# Autodesk Inventor assembly: 20-J2
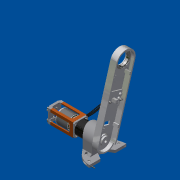
[picture p0: Inventor's stored thumbnail of the model, 180x180]
Saved by Autodesk Inventor 2018 (Build 220112000, 112)
## iProperties
Created: 2020-01-14
Part Number: 20-J2
Document SubType Name: Assembly
Designer: Bunny320
Author: Bunny320
## Documents named in this file (10)
- C:\Users\Bunny320\Desktop\sechs\4-CAD\20-J2.iam
- C:\Users\Bunny320\Desktop\sechs\4-CAD\201-flange-with motor.ipt
- C:\Users\Bunny320\Desktop\sechs\4-CAD\standardParts\61807-2RS1\61807-2RS1.iam
- C:\Users\Bunny320\Desktop\sechs\4-CAD\motor unit.iam
- C:\Users\Bunny320\Desktop\sechs\4-CAD\203-link left.ipt
- C:\Users\Bunny320\Desktop\sechs\4-CAD\standardParts\W 638_3-2Z\W 638_3-2Z.iam
- C:\Users\Bunny320\Documents\Inventor\Content Center Files\R2018\en-US\ISO 10642(2)\ISO 10642  - M4  x  20.ipt
- C:\Users\Bunny320\Documents\Inventor\Content Center Files\R2018\en-US\ISO 4762(1)\DIN EN ISO 4762 - M3 x 12.ipt
- C:\Users\Bunny320\Documents\Inventor\Content Center Files\R2018\en-US\ISO 4762(1)\DIN EN ISO 4762 - M3 x 20.ipt
- C:\Users\Bunny320\Documents\Inventor\Content Center Files\R2018\en-US\DIN EN ISO 4032\DIN EN ISO 4032 - M3.ipt
## Components (19 placed, 9 different names)
1. 201-flange-with motor:1 — Flush:1, Flush:2, Flush:3, Mate:3, Mate:4, Mate:7, Mate:8, Mate:9, Mate:21, Mate:22, Mate:23, Mate:24, Mate:31, Mate:32, Mate:33, Mate:34, Mate:35, Mate:36, Mate:37, Mate:38, Mate:39, Mate:40, Mate:41, Mate:42
2. 61807-2RS1:1 [sub-assembly] — Mate:3, Mate:4, Mate:14
3. motor unit:1 [sub-assembly] — Mate:7, Mate:8, Mate:9, Mate:13
4. 203-link left:1 — Mate:13, Mate:14, Mate:15, Mate:16, Mate:17, Mate:18, Mate:19, Mate:20, Mate:25, Mate:29
5. 61807-2RS1:3 [sub-assembly] — Mate:15, Mate:16
6. W 638_3-2Z:1 [sub-assembly] — Mate:17, Mate:20, Mate:26, Mate:30
7. W 638_3-2Z:2 [sub-assembly] — Mate:18, Mate:19
8. DIN EN ISO 10642 M4  x  20:1 — Mate:21
9. DIN EN ISO 10642 M4  x  20:2 — Mate:22
10. DIN EN ISO 10642 M4  x  20:3 — Mate:23
11. DIN EN ISO 10642 M4  x  20:4 — Mate:24
12. DIN EN ISO 4762 M3 x 12:1 — Mate:25, Mate:26
13. DIN EN ISO 4762 M3 x 12:3 — Mate:29, Mate:30
14. DIN EN ISO 4762 M3 x 12:4 — Mate:31, Mate:32
15. DIN EN ISO 4762 M3 x 12:5 — Mate:33, Mate:34
16. DIN EN ISO 4762 M3 x 12:6 — Mate:35, Mate:36
17. DIN EN ISO 4762 M3 x 12:7 — Mate:37, Mate:38
18. DIN EN ISO 4762 M3 x 20:1 — Mate:39, Mate:40
19. DIN EN ISO 4032 M3:1 — Mate:41, Mate:42
## Relationships (36: Mate 33, Flush 3)
- Flush:1: 201-flange-with motor:1
- Flush:2: 201-flange-with motor:1
- Flush:3: 201-flange-with motor:1
- Mate:3: 201-flange-with motor:1 ↔ 61807-2RS1:1
- Mate:4: 201-flange-with motor:1 ↔ 61807-2RS1:1
- Mate:7: 201-flange-with motor:1 ↔ motor unit:1
- Mate:8: 201-flange-with motor:1 ↔ motor unit:1
- Mate:9: 201-flange-with motor:1 ↔ motor unit:1
- Mate:13: motor unit:1 ↔ 203-link left:1
- Mate:14: 61807-2RS1:1 ↔ 203-link left:1
- Mate:15: 203-link left:1 ↔ 61807-2RS1:3
- Mate:16: 203-link left:1 ↔ 61807-2RS1:3
- Mate:17: 203-link left:1 ↔ W 638_3-2Z:1
- Mate:18: 203-link left:1 ↔ W 638_3-2Z:2
- Mate:19: 203-link left:1 ↔ W 638_3-2Z:2
- Mate:20: 203-link left:1 ↔ W 638_3-2Z:1
- Mate:21: 201-flange-with motor:1 ↔ DIN EN ISO 10642 M4  x  20:1
- Mate:22: 201-flange-with motor:1 ↔ DIN EN ISO 10642 M4  x  20:2
- Mate:23: 201-flange-with motor:1 ↔ DIN EN ISO 10642 M4  x  20:3
- Mate:24: 201-flange-with motor:1 ↔ DIN EN ISO 10642 M4  x  20:4
- Mate:25: 203-link left:1 ↔ DIN EN ISO 4762 M3 x 12:1
- Mate:26: W 638_3-2Z:1 ↔ DIN EN ISO 4762 M3 x 12:1
- Mate:29: 203-link left:1 ↔ DIN EN ISO 4762 M3 x 12:3
- Mate:30: W 638_3-2Z:1 ↔ DIN EN ISO 4762 M3 x 12:3
- Mate:31: 201-flange-with motor:1 ↔ DIN EN ISO 4762 M3 x 12:4
- Mate:32: 201-flange-with motor:1 ↔ DIN EN ISO 4762 M3 x 12:4
- Mate:33: 201-flange-with motor:1 ↔ DIN EN ISO 4762 M3 x 12:5
- Mate:34: 201-flange-with motor:1 ↔ DIN EN ISO 4762 M3 x 12:5
- Mate:35: 201-flange-with motor:1 ↔ DIN EN ISO 4762 M3 x 12:6
- Mate:36: 201-flange-with motor:1 ↔ DIN EN ISO 4762 M3 x 12:6
- Mate:37: 201-flange-with motor:1 ↔ DIN EN ISO 4762 M3 x 12:7
- Mate:38: 201-flange-with motor:1 ↔ DIN EN ISO 4762 M3 x 12:7
- Mate:39: 201-flange-with motor:1 ↔ DIN EN ISO 4762 M3 x 20:1
- Mate:40: 201-flange-with motor:1 ↔ DIN EN ISO 4762 M3 x 20:1
- Mate:41: 201-flange-with motor:1 ↔ DIN EN ISO 4032 M3:1
- Mate:42: 201-flange-with motor:1 ↔ DIN EN ISO 4032 M3:1
